# Autodesk Inventor assembly: PrismMountCube
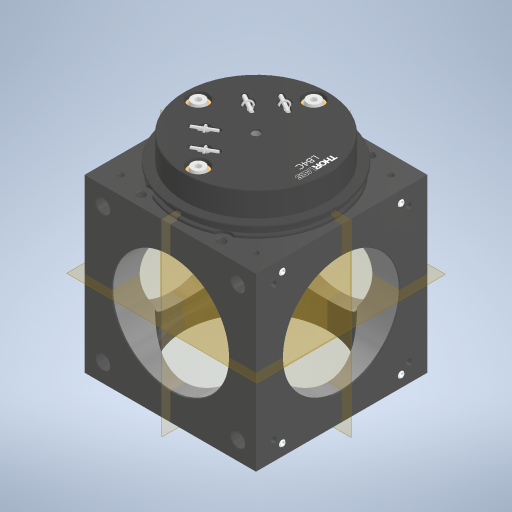
[picture p0: Inventor's stored thumbnail of the model, 512x512]
Saved by Autodesk Inventor 2023 (Build 270158000, 158)
## iProperties
Created: 2024-01-10
Part Number: PrismMountCube
Document SubType Name: Assembly
Designer: kerlin
Author: kerlin
## Documents named in this file (4)
- C:\Users\kerlin\Documents\KerlinLab\KTN\Multipass\MechanicalDrawing\PrismMountCube.iam
- C:\Users\kerlin\Downloads\LC6W-Solidworks.ipt
- C:\Users\kerlin\Downloads\MRA03-P01-Solidworks.ipt
- C:\Users\kerlin\Documents\KerlinLab\KTN\Multipass\MechanicalDrawing\LB4C-Solidworks.ipt
## Components (3 placed, 3 different names)
1. LC6W-Solidworks:1 — Flush:1, Mate:1, Mate:2, Mate:3, Mate:4
2. MRA03-P01-Solidworks:1 — Flush:1, Mate:1, Mate:2
3. LB4C-Solidworks:1 — Mate:3, Mate:4
## Relationships (5: Mate 4, Flush 1)
- Flush:1: LC6W-Solidworks:1 ↔ MRA03-P01-Solidworks:1
- Mate:1: LC6W-Solidworks:1 ↔ MRA03-P01-Solidworks:1
- Mate:2: LC6W-Solidworks:1 ↔ MRA03-P01-Solidworks:1
- Mate:3: LC6W-Solidworks:1 ↔ LB4C-Solidworks:1
- Mate:4: LC6W-Solidworks:1 ↔ LB4C-Solidworks:1
